# Autodesk Inventor assembly: Skystone Arm
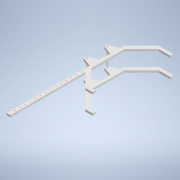
[picture p0: Inventor's stored thumbnail of the model, 180x180]
Saved by Autodesk Inventor 2020 (Build 240168000, 168)
## iProperties
Created: 2020-02-26
Part Number: Skystone Arm
Document SubType Name: Assembly
Designer: shrey
Author: shrey
## Documents named in this file (4)
- C:\Users\shrey\OneDrive\Documents\Skystone Arm.iam
- C:\Users\shrey\OneDrive\Documents\Arm.ipt
- C:\Users\shrey\OneDrive\Documents\Connector.ipt
- C:\Users\shrey\OneDrive\Documents\ServoArm.ipt
## Components (5 placed, 4 different names)
1. Clasp: 1 — Flush:1, Mate:1, Flush:2, Mate:2, Mate:4
2. Clasp: 2
3. Connector:1 — Flush:2, Mate:2
4. Connector:2 — Flush:1, Mate:1, Mate:3
5. ServoArm:1 — Mate:3, Mate:4
## Relationships (6: Mate 4, Flush 2)
- Flush:1 (-3.175 mm): Clasp: 1 ↔ Connector:2
- Mate:1: Clasp: 1 ↔ Connector:2
- Flush:2 (-3.175 mm): Clasp: 1 ↔ Connector:1
- Mate:2: Clasp: 1 ↔ Connector:1
- Mate:3: Connector:2 ↔ ServoArm:1
- Mate:4 (22.225 mm): Clasp: 1 ↔ ServoArm:1
